# Autodesk Inventor assembly: LegEnd
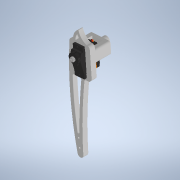
[picture p0: Inventor's stored thumbnail of the model, 180x180]
Saved by Autodesk Inventor 2020.3 (Build 243373000, 373)
## iProperties
Created: 2022-03-31
Part Number: LegEnd
Document SubType Name: Assembly
Designer: sanyi
Author: sanyi
## Documents named in this file (4)
- C:\Users\sanyi\Documents\Inventor\Quadropod\Quadropod MDL\SimulationModell_Assembly\LegEnd.iam
- C:\Users\sanyi\Documents\Inventor\Quadropod\LegEnd_Right_v2.ipt
- C:\Users\sanyi\Documents\Inventor\Quadropod\LegPin_v1.ipt
- C:\Users\sanyi\Documents\Inventor\Quadropod\SH-0257MG.ipt
## Components (3 placed, 3 different names)
1. LegEnd_Right_v2:1 — Insert:1, Insert:2, Insert:3, Angle:1, Mate:1, Mate:2, Mate:3
2. LegPin_v1:1 — Insert:1, Insert:2
3. SH-0257MG:1 — Insert:3, Angle:1
## Relationships (7: Insert 3, Mate 3, Angle 1)
- Insert:1: LegEnd_Right_v2:1 ↔ LegPin_v1:1
- Insert:2: LegEnd_Right_v2:1 ↔ LegPin_v1:1
- Insert:3: LegEnd_Right_v2:1 ↔ SH-0257MG:1
- Angle:1 (0 deg): LegEnd_Right_v2:1 ↔ SH-0257MG:1
- Mate:1: LegEnd_Right_v2:1
- Mate:2: LegEnd_Right_v2:1
- Mate:3: LegEnd_Right_v2:1
